# Autodesk Inventor assembly: Assembly1
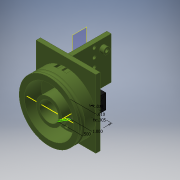
[picture p0: Inventor's stored thumbnail of the model, 180x180]
Saved by Autodesk Inventor 2018 (Build 220112000, 112)
## iProperties
Created: 2018-01-26
Part Number: Assembly1
Document SubType Name: Assembly
Designer: prakh
Author: prakh
## Documents named in this file (4)
- D:\GIT\ModernMobility\CADS\Alternate Wheel\Assembly1.iam
- D:\GIT\ModernMobility\CADS\Alternate Wheel\mounting plate.ipt
- D:\GIT\ModernMobility\CADS\Alternate Wheel\motor mount 2.ipt
- D:\GIT\ModernMobility\CADS\Alternate Wheel\Imported Components\microServo-sg90\microServo-sg90.ipt
## Components (3 placed, 3 different names)
1. mounting plate:1 — Mate:1, Mate:2, Mate:3, Mate:4, Mate:5, Mate:6, Angle:1
2. motor mount 2:1 — Mate:1, Mate:2, Mate:3
3. microServo-sg90:1 — Mate:4, Mate:5, Mate:6, Angle:1
## Relationships (7: Mate 6, Angle 1)
- Mate:1: mounting plate:1 ↔ motor mount 2:1
- Mate:2: mounting plate:1 ↔ motor mount 2:1
- Mate:3: mounting plate:1 ↔ motor mount 2:1
- Mate:4: mounting plate:1 ↔ microServo-sg90:1
- Mate:5: mounting plate:1 ↔ microServo-sg90:1
- Mate:6: mounting plate:1 ↔ microServo-sg90:1
- Angle:1 (0 deg): mounting plate:1 ↔ microServo-sg90:1
